# Autodesk Inventor assembly: Geneva2
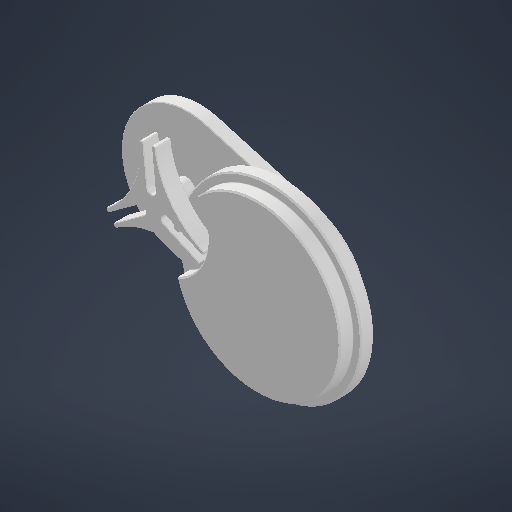
[picture p0: Inventor's stored thumbnail of the model, 512x512]
Saved by Autodesk Inventor 2026.3 (Build 303398000, 398)
## iProperties
Created: 2026-05-01
Part Number: Geneva2
Document SubType Name: Assembly
Designer: frede
Author: frede
## Documents named in this file (4)
- E:\Git\AppliedAutomationProject\feeder\trayFeeder\step\Geneva2.iam
- E:\Git\AppliedAutomationProject\feeder\trayFeeder\Geneva2_Output.ipt
- E:\Git\AppliedAutomationProject\feeder\trayFeeder\Geneva2_Input.ipt
- E:\Git\AppliedAutomationProject\feeder\trayFeeder\Geneva2_BasePlate.ipt
## Components (3 placed, 3 different names)
1. Geneva2_Output:1 — Mate:5, Mate:6, Mate:7
2. Geneva2_Input:1 — Mate:1, Mate:4, Mate:7
3. Geneva2_BasePlate:1 — Mate:1, Mate:4, Mate:5, Mate:6
## Relationships (5: Mate 5)
- Mate:1: Geneva2_Input:1 ↔ Geneva2_BasePlate:1
- Mate:4: Geneva2_Input:1 ↔ Geneva2_BasePlate:1
- Mate:5: Geneva2_Output:1 ↔ Geneva2_BasePlate:1
- Mate:6: Geneva2_Output:1 ↔ Geneva2_BasePlate:1
- Mate:7 (1.6 mm): Geneva2_Output:1 ↔ Geneva2_Input:1
